# Autodesk Inventor assembly: assembly_pinball_plunger_handle
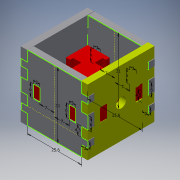
[picture p0: Inventor's stored thumbnail of the model, 180x180]
Saved by Autodesk Inventor 2017 (Build 210142000, 142)
## iProperties
Created: 2017-01-19
Part Number: assembly_pinball_plunger_handle
Document SubType Name: Assembly
Designer: John
Author: John
## Documents named in this file (4)
- C:\Users\John\Dropbox\ECE115\pinball-project\plunger\assembly_pinball_plunger_handle.iam
- C:\Users\John\Desktop\plunger_handle_center.ipt
- C:\Users\John\Desktop\part_plunger_handle_side1.ipt
- C:\Users\John\Desktop\part_plunger_handle_side2.ipt
## Components (5 placed, 3 different names)
1. plunger_handle_center:1 — Mate:1, Flush:1, Flush:2, Flush:10
2. part_plunger_handle_side1:1 — Mate:1, Flush:1, Flush:2, Mate:2, Mate:3, Flush:5, Flush:8, Flush:9, Flush:10
3. part_plunger_handle_side2:1 — Mate:2, Flush:6, Flush:7, Flush:8
4. part_plunger_handle_side2:2 — Mate:3, Mate:4, Flush:3, Flush:4, Flush:5, Flush:9
5. part_plunger_handle_side1:2 — Mate:4, Flush:3, Flush:4, Flush:6, Flush:7
## Relationships (14: Flush 10, Mate 4)
- Mate:1: plunger_handle_center:1 ↔ part_plunger_handle_side1:1
- Flush:1: plunger_handle_center:1 ↔ part_plunger_handle_side1:1
- Flush:2: plunger_handle_center:1 ↔ part_plunger_handle_side1:1
- Mate:2: part_plunger_handle_side1:1 ↔ part_plunger_handle_side2:1
- Mate:3: part_plunger_handle_side1:1 ↔ part_plunger_handle_side2:2
- Mate:4: part_plunger_handle_side2:2 ↔ part_plunger_handle_side1:2
- Flush:3: part_plunger_handle_side2:2 ↔ part_plunger_handle_side1:2
- Flush:4: part_plunger_handle_side2:2 ↔ part_plunger_handle_side1:2
- Flush:5: part_plunger_handle_side1:1 ↔ part_plunger_handle_side2:2
- Flush:6: part_plunger_handle_side2:1 ↔ part_plunger_handle_side1:2
- Flush:7: part_plunger_handle_side2:1 ↔ part_plunger_handle_side1:2
- Flush:8: part_plunger_handle_side1:1 ↔ part_plunger_handle_side2:1
- Flush:9: part_plunger_handle_side1:1 ↔ part_plunger_handle_side2:2
- Flush:10: plunger_handle_center:1 ↔ part_plunger_handle_side1:1
